# Autodesk Inventor assembly: pulley
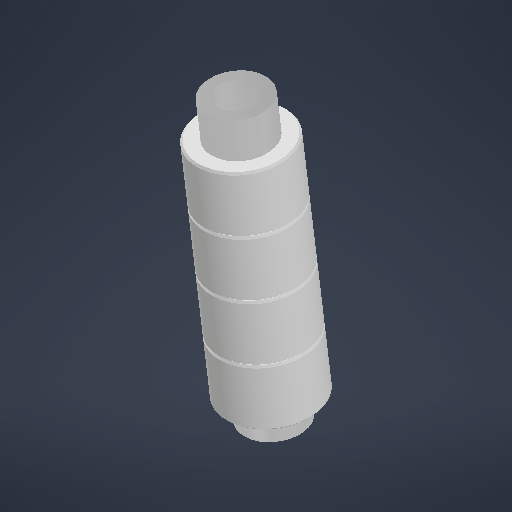
[picture p0: Inventor's stored thumbnail of the model, 512x512]
Saved by Autodesk Inventor 2026.1 (Build 301233000, 233)
## iProperties
Created: 2026-05-27
Part Number: pulley
Document SubType Name: Assembly
Designer: aaron
Author: aaron
## Documents named in this file (3)
- D:\work\loopandpixel\openworkoutsystem\cad\v5\pulley.iam
- D:\work\loopandpixel\openworkoutsystem\cad\v5\bearings\bearing_12x8x8.ipt
- D:\work\loopandpixel\openworkoutsystem\cad\v5\M5x40mm_coupler.ipt
## Components (5 placed, 2 different names)
1. bearing_12x8x8:1 — Mate:1, Insert:1
2. M5x40mm_coupler:1 — Mate:1
3. bearing_12x8x8:2 — Insert:1, Insert:2
4. bearing_12x8x8:3 — Insert:2, Insert:3
5. bearing_12x8x8:4 — Insert:3
## Relationships (4: Insert 3, Mate 1)
- Mate:1: bearing_12x8x8:1 ↔ M5x40mm_coupler:1
- Insert:1: bearing_12x8x8:1 ↔ bearing_12x8x8:2
- Insert:2: bearing_12x8x8:2 ↔ bearing_12x8x8:3
- Insert:3: bearing_12x8x8:3 ↔ bearing_12x8x8:4
